# Autodesk Inventor assembly: 8020_structure
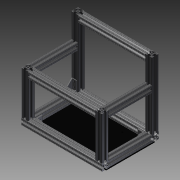
[picture p0: Inventor's stored thumbnail of the model, 180x180]
Saved by Autodesk Inventor 2015 (Build 190159000, 159)
## iProperties
Created: 2017-04-21
Part Number: 8020_structure
Document SubType Name: Assembly
Designer: Raghava
Author: Raghava
## Documents named in this file (8)
- C:\Users\Raghava\Desktop\jackal_model\8020 Components\8020_structure.iam
- C:\Users\Raghava\Desktop\jackal_model\8020 Components\1010_with_tnut.iam
- C:\Users\Raghava\Desktop\jackal_model\Base Plate.ipt
- C:\Users\Raghava\Desktop\jackal_model\8020 Components\1010_299_4mm.ipt
- C:\Users\Raghava\Desktop\jackal_model\8020 Components\4119.ipt
- C:\Users\Raghava\Desktop\jackal_model\8020 Components\1010_160mm.ipt
- C:\Users\Raghava\Desktop\jackal_model\8020 Components\14058_m.ipt
- C:\Users\Raghava\Desktop\jackal_model\8020 Components\1010_248_6mm.ipt
## Components (18 placed, 7 different names)
1. 1010_with_tnut:1 [sub-assembly] — Mate:1, Flush:1, Flush:2, Mate:7, Mate:10, Flush:3, Flush:4, Mate:18, Mate:20
2. 1010_with_tnut:2 [sub-assembly] — Mate:2, Flush:1, Flush:2, Mate:6, Mate:8, Mate:9, Mate:14, Mate:16, Mate:30, Mate:36
3. Base Plate:1 — Mate:4, Mate:5, Mate:8, Mate:11, Mate:12, Mate:21, Mate:22, Mate:23, Mate:24
4. 1010_299_4mm:1 — Mate:9, Flush:3, Mate:11, Mate:15, Mate:17, Flush:9, Flush:10, Flush:11, Flush:12, Mate:27, Mate:28
5. 1010_299_4mm:2 — Mate:10, Flush:4, Mate:12, Mate:13, Mate:19, Flush:17, Flush:18, Flush:19, Flush:20, Mate:31, Mate:32
6. 4119:1 — Mate:13, Mate:14, Mate:21
7. 4119:2 — Mate:15, Mate:16, Mate:22
8. 4119:3 — Mate:17, Mate:18, Mate:23
9. 4119:4 — Mate:19, Mate:20, Mate:24
10. 1010_160mm:1 — Flush:9, Flush:10, Mate:27, Flush:15, Flush:22, Mate:34, Flush:23
11. 1010_160mm:2 — Flush:11, Flush:12, Mate:28, Flush:16, Flush:21, Mate:37
12. 14058_m:1 — Mate:30, Mate:35, Mate:36
13. 1010_160mm:3 — Flush:15, Flush:22, Mate:34
14. 1010_160mm:4 — Flush:16, Flush:21, Mate:33
15. 1010_248_6mm:1 — Flush:19, Flush:20, Mate:32, Mate:35, Mate:38, Flush:24
16. 1010_248_6mm:2 — Flush:17, Flush:18, Mate:31, Mate:33
17. 1010_248_6mm:3 — Mate:38, Flush:24
18. 1010_248_6mm:4 — Flush:23, Mate:37
## Relationships (53: Mate 35, Flush 18)
- Mate:1: 1010_with_tnut:1
- Mate:2: 1010_with_tnut:2
- Flush:1: 1010_with_tnut:1 ↔ 1010_with_tnut:2
- Mate:3 (274 mm)
- Flush:2: 1010_with_tnut:1 ↔ 1010_with_tnut:2
- Mate:4: Base Plate:1
- Mate:5: Base Plate:1
- Mate:6: 1010_with_tnut:2
- Mate:7: 1010_with_tnut:1
- Mate:8: 1010_with_tnut:2 ↔ Base Plate:1
- Mate:9: 1010_with_tnut:2 ↔ 1010_299_4mm:1
- Mate:10: 1010_with_tnut:1 ↔ 1010_299_4mm:2
- Flush:3: 1010_with_tnut:1 ↔ 1010_299_4mm:1
- Flush:4: 1010_with_tnut:1 ↔ 1010_299_4mm:2
- Mate:11: Base Plate:1 ↔ 1010_299_4mm:1
- Mate:12: Base Plate:1 ↔ 1010_299_4mm:2
- Mate:13: 1010_299_4mm:2 ↔ 4119:1
- Mate:14: 1010_with_tnut:2 ↔ 4119:1
- Mate:15: 1010_299_4mm:1 ↔ 4119:2
- Mate:16: 1010_with_tnut:2 ↔ 4119:2
- Mate:17: 1010_299_4mm:1 ↔ 4119:3
- Mate:18: 1010_with_tnut:1 ↔ 4119:3
- Mate:19: 1010_299_4mm:2 ↔ 4119:4
- Mate:20: 1010_with_tnut:1 ↔ 4119:4
- Mate:21: Base Plate:1 ↔ 4119:1
- Mate:22: Base Plate:1 ↔ 4119:2
- Mate:23: Base Plate:1 ↔ 4119:3
- Mate:24: Base Plate:1 ↔ 4119:4
- Flush:9: 1010_299_4mm:1 ↔ 1010_160mm:1
- Flush:10: 1010_299_4mm:1 ↔ 1010_160mm:1
- Flush:11: 1010_299_4mm:1 ↔ 1010_160mm:2
- Flush:12: 1010_299_4mm:1 ↔ 1010_160mm:2
- Mate:27: 1010_299_4mm:1 ↔ 1010_160mm:1
- Mate:28: 1010_299_4mm:1 ↔ 1010_160mm:2
- Mate:30: 1010_with_tnut:2 ↔ 14058_m:1
- Flush:15: 1010_160mm:1 ↔ 1010_160mm:3
- Flush:16: 1010_160mm:2 ↔ 1010_160mm:4
- Flush:17: 1010_299_4mm:2 ↔ 1010_248_6mm:2
- Flush:18: 1010_299_4mm:2 ↔ 1010_248_6mm:2
- Flush:19: 1010_299_4mm:2 ↔ 1010_248_6mm:1
- Flush:20: 1010_299_4mm:2 ↔ 1010_248_6mm:1
- Mate:31: 1010_299_4mm:2 ↔ 1010_248_6mm:2
- Mate:32: 1010_299_4mm:2 ↔ 1010_248_6mm:1
- Flush:21: 1010_160mm:2 ↔ 1010_160mm:4
- Mate:33: 1010_160mm:4 ↔ 1010_248_6mm:2
- Flush:22: 1010_160mm:1 ↔ 1010_160mm:3
- Mate:34: 1010_160mm:1 ↔ 1010_160mm:3
- Mate:35: 14058_m:1 ↔ 1010_248_6mm:1
- Mate:36 (1 mm): 1010_with_tnut:2 ↔ 14058_m:1
- Flush:23: 1010_160mm:1 ↔ 1010_248_6mm:4
- Mate:37: 1010_160mm:2 ↔ 1010_248_6mm:4
- Mate:38: 1010_248_6mm:1 ↔ 1010_248_6mm:3
- Flush:24: 1010_248_6mm:1 ↔ 1010_248_6mm:3
